# Autodesk Inventor assembly: Assembly
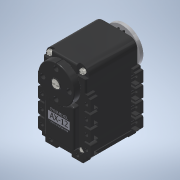
[picture p0: Inventor's stored thumbnail of the model, 180x180]
Saved by Autodesk Inventor 2021 (Build 250183000, 183)
## iProperties
Created: 2019-11-04
Part Number: Assembly
Document SubType Name: Assembly
Designer: izuwa
Author: izuwa
## Documents named in this file (3)
- C:\Users\izuwa\Documents\Inventor\AX-12 SERVO MOTOR\Assembly.iam
- C:\Users\izuwa\Documents\Inventor\ironSpidey\ax-12.ipt
- C:\Users\izuwa\Documents\Inventor\ironSpidey\B11.ipt
## Components (2 placed, 2 different names)
1. ax-12:1 — Insert:1
2. B11:1 — Insert:1
## Relationships (1: Insert 1)
- Insert:1: ax-12:1 ↔ B11:1
